# Autodesk Inventor assembly: wahacz_tylny_final
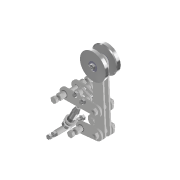
[picture p0: Inventor's stored thumbnail of the model, 180x180]
Saved by Autodesk Inventor 2020.3 (Build 243373000, 373)
## iProperties
Created: 2021-10-24
Part Number: wahacz_tylny_final
Document SubType Name: Assembly
Designer: patry
Author: patry
## Documents named in this file (25)
- C:\Users\patry\Desktop\Semestr 7\Inzynierka\Projekt inventor\Ariadna_inzynierka\Workspaces\Obszar roboczy\Obszar roboczy\Naped\Zawieszenie_v3\wahacz_tylny_final.iam
- C:\Users\patry\Desktop\Semestr 7\Inzynierka\Projekt inventor\Ariadna_inzynierka\Workspaces\Obszar roboczy\Obszar roboczy\Naped\Zawieszenie_v3\ramie_1_wahacza.ipt
- C:\Users\patry\Desktop\Semestr 7\Inzynierka\Projekt inventor\Ariadna_inzynierka\Workspaces\Obszar roboczy\Obszar roboczy\Naped\Zawieszenie_v3\tuleja_TUF106040.ipt
- C:\Users\patry\Desktop\Semestr 7\Inzynierka\Projekt inventor\Ariadna_inzynierka\Workspaces\Obszar roboczy\Obszar roboczy\Naped\Sruby\M6_nut_5mm.ipt
- C:\Users\patry\Desktop\Semestr 7\Inzynierka\Projekt inventor\Ariadna_inzynierka\Workspaces\Obszar roboczy\Obszar roboczy\Naped\Amortyzator\Korpus.ipt
- C:\Users\patry\Desktop\Semestr 7\Inzynierka\Projekt inventor\Ariadna_inzynierka\Workspaces\Obszar roboczy\Obszar roboczy\Naped\Amortyzator\Tlok.ipt
- C:\Users\patry\Desktop\Semestr 7\Inzynierka\Projekt inventor\Ariadna_inzynierka\Workspaces\Obszar roboczy\Obszar roboczy\Naped\Amortyzator\Nakretka.ipt
- C:\Users\patry\Desktop\Semestr 7\Inzynierka\Projekt inventor\Ariadna_inzynierka\Workspaces\Obszar roboczy\Obszar roboczy\Naped\Sruby\M5_nut_5mm.ipt
- C:\Users\patry\Desktop\Semestr 7\Inzynierka\Projekt inventor\Ariadna_inzynierka\Workspaces\Obszar roboczy\Obszar roboczy\Naped\Sruby\M5_70_shaft.ipt
- C:\Users\patry\Desktop\Semestr 7\Inzynierka\Projekt inventor\Ariadna_inzynierka\Workspaces\Obszar roboczy\Obszar roboczy\Naped\Sruby\M3_16_shaft.ipt
- C:\Users\patry\Desktop\Semestr 7\Inzynierka\Projekt inventor\Ariadna_inzynierka\Workspaces\Obszar roboczy\Obszar roboczy\Naped\Sruby\M3_nut_2,5mm.ipt
- C:\Users\patry\Desktop\Semestr 7\Inzynierka\Projekt inventor\Ariadna_inzynierka\Workspaces\Obszar roboczy\Obszar roboczy\Naped\Zawieszenie_v3\wspornik_amortyzatora.ipt
- C:\Users\patry\Desktop\Semestr 7\Inzynierka\Projekt inventor\Ariadna_inzynierka\Workspaces\Obszar roboczy\Obszar roboczy\Naped\Sruby\M6_40_shaft.ipt
- C:\Users\patry\Desktop\Semestr 7\Inzynierka\Projekt inventor\Ariadna_inzynierka\Workspaces\Obszar roboczy\Obszar roboczy\Naped\Sruby\tuleja_M6_M10_7.ipt
- C:\Users\patry\Desktop\Semestr 7\Inzynierka\Projekt inventor\Ariadna_inzynierka\Workspaces\Obszar roboczy\Obszar roboczy\Naped\Sruby\M6_1,25_pad.ipt
- C:\Users\patry\Desktop\Semestr 7\Inzynierka\Projekt inventor\Ariadna_inzynierka\Workspaces\Obszar roboczy\Obszar roboczy\Naped\Sruby\M6_70_shaft.ipt
- C:\Users\patry\Desktop\Semestr 7\Inzynierka\Projekt inventor\Ariadna_inzynierka\Workspaces\Obszar roboczy\Obszar roboczy\Naped\Sruby\M5_40_shaft.ipt
- M5_shaft.ipt
- C:\Users\patry\Desktop\Semestr 7\Inzynierka\Projekt inventor\Ariadna_inzynierka\Workspaces\Obszar roboczy\Obszar roboczy\Naped\Sruby\tuleja_M5_M9_4,5.ipt
- C:\Users\patry\Desktop\Semestr 7\Inzynierka\Projekt inventor\Ariadna_inzynierka\Workspaces\Obszar roboczy\Obszar roboczy\Naped\Zawieszenie_v3\glowny_wahacz_zewn.ipt
- C:\Users\patry\Desktop\Semestr 7\Inzynierka\Projekt inventor\Ariadna_inzynierka\Workspaces\Obszar roboczy\Obszar roboczy\Naped\Zawieszenie_v3\independent_wheel_pair.iam
- C:\Users\patry\Desktop\Semestr 7\Inzynierka\Projekt inventor\Ariadna_inzynierka\Workspaces\Obszar roboczy\Obszar roboczy\Naped\Sruby\tuleja_M6_M10_6.ipt
- C:\Users\patry\Desktop\Semestr 7\Inzynierka\Projekt inventor\Ariadna_inzynierka\Workspaces\Obszar roboczy\Obszar roboczy\Naped\Sruby\tuleja_M5_M9_17.5.ipt
- C:\Users\patry\Desktop\Semestr 7\Inzynierka\Projekt inventor\Ariadna_inzynierka\Workspaces\Obszar roboczy\Obszar roboczy\Naped\Zawieszenie_v3\ramie_2_wahacza_tylnego.ipt
- C:\Users\patry\Desktop\Semestr 7\Inzynierka\Projekt inventor\Ariadna_inzynierka\Workspaces\Obszar roboczy\Obszar roboczy\Naped\Sruby\M6x25_plaski_leb.ipt
## Components (72 placed, 23 different names)
1. ramie_1_wahacza:1 — Zestawiające:7, Zestawiające:8, Kątowe:4, Zestawiające:108, Zestawiające:109, Zestawiające:110, Równoległe:6, Zestawiające:114, Zestawiające:158, Równoległe:11, Zestawiające:159, Równoległe:12, Zestawiające:161, Zestawiające:163, Zestawiające:175, Zestawiające:179, Zestawiające:203, Zestawiające:204
2. tuleja_TUF106040:1 — Zestawiające:93, Zestawiające:200, Zestawiające:250, Zestawiające:251
3. tuleja_TUF106040:2 — Zestawiające:238, Zestawiające:252, Zestawiające:253, Zestawiające:257, Zestawiające:267
4. tuleja_TUF106040:3 — Zestawiające:202, Zestawiające:203, Zestawiające:204
5. tuleja_TUF106040:4 — Zestawiające:7, Zestawiające:8, Kątowe:4, Zestawiające:111, Zestawiające:132
6. tuleja_TUF106040:5 — Zestawiające:89, Zestawiające:201, Zestawiające:240
7. tuleja_TUF106040:6 — Zestawiające:88, Zestawiające:90, Zestawiające:189, Zestawiające:198
8. tuleja_TUF106040:7 — Zestawiające:93, Zestawiające:112, Zestawiające:140, Zestawiające:258, Zestawiające:259
9. tuleja_TUF106040:8 — Zestawiające:236, Zestawiające:260, Zestawiające:261, Zestawiające:262
10. M6_nut_5mm:2 — Zestawiające:113, Zestawiające:114
11. Korpus:1 — Walcowe:1, Zestawiające:83, Równoległe:4, Zestawiające:87, Zestawiające:248
12. Tlok:1 — Walcowe:1, Zestawiające:102, Zestawiające:103
13. Nakretka:1
14. M5_nut_5mm:1 — Zestawiające:84, Zestawiające:86, Zestawiające:87, Równoległe:9, Równoległe:10, Zestawiające:242
15. M5_70_shaft:1 — Zestawiające:83, Równoległe:4, Zestawiające:84, Zestawiające:85, Równoległe:8, Zestawiające:241, Zestawiające:243, Zestawiające:245, Zestawiające:247
16. ramie_1_wahacza:3 — Zestawiające:88, Zestawiające:89, Zestawiające:90, Zestawiające:116, Zestawiające:165, Zestawiające:167, Zestawiające:173, Zestawiające:177, Zestawiające:201, Zestawiające:224
17. M5_nut_5mm:2 — Zestawiające:85, Zestawiające:86, Zestawiające:244
18. M3_16_shaft:1 — Zestawiające:97, Równoległe:5, Zestawiające:98, Zestawiające:100, Zestawiające:102
19. M3_nut_2,5mm:1 — Zestawiające:98, Zestawiające:99
20. M3_nut_2,5mm:2 — Zestawiające:100, Zestawiające:101
21. wspornik_amortyzatora:1 — Zestawiające:94, Zestawiające:95, Zestawiające:96, Równoległe:5, Zestawiające:99, Zestawiające:108, Zestawiające:109, Zestawiające:110
22. wspornik_amortyzatora:2 — Zestawiające:94, Zestawiające:95, Zestawiające:96, Zestawiające:97, Zestawiające:101, Zestawiające:103
23. M6_40_shaft:1 — Zestawiające:111, Równoległe:6, Zestawiające:113, Zestawiające:115, Zestawiające:121, Zestawiające:127, Zestawiające:131, Zestawiające:182, Zestawiające:186, Zestawiające:189
24. M6_40_shaft:2 — Zestawiające:112, Zestawiające:117, Zestawiające:119, Zestawiające:123, Zestawiające:135, Zestawiające:139, Zestawiające:180, Zestawiające:185, Równoległe:13
25. M6_nut_5mm:11 — Zestawiające:115, Zestawiające:116
26. M6_nut_5mm:12 — Zestawiające:117, Zestawiające:270, Równoległe:13
27. M6_nut_5mm:13 — Zestawiające:119, Zestawiające:269
28. tuleja_M6_M10_7:1 — Zestawiające:121, Zestawiające:196
29. tuleja_M6_M10_7:2 — Zestawiające:123, Zestawiające:181
30. M6_1,25_pad:1 — Zestawiające:125, Zestawiające:126, Zestawiające:127, Zestawiające:197
31. M6_1,25_pad:2 — Zestawiające:125, Zestawiające:126, Zestawiające:198
32. M6_1,25_pad:3 — Zestawiające:131, Zestawiające:132
33. M6_1,25_pad:4 — Zestawiające:194
34. M6_1,25_pad:5 — Zestawiające:135, Zestawiające:199
35. M6_1,25_pad:6 — Zestawiające:200
36. M6_1,25_pad:7 — Zestawiające:139, Zestawiające:140
37. M6_1,25_pad:8 — Zestawiające:195
38. M6_70_shaft:2 — Równoległe:8, Zestawiające:144, Zestawiające:145, Zestawiające:202, Zestawiające:229, Zestawiające:231, Zestawiające:233, Zestawiające:239
39. M6_nut_5mm:14 — Zestawiające:144, Zestawiające:146, Zestawiające:230
40. M6_nut_5mm:15 — Zestawiające:145, Zestawiające:146, Równoległe:9, Zestawiające:232
41. M6_nut_5mm:16 — Zestawiające:148, Zestawiające:228, Zestawiające:264
42. M6_nut_5mm:17 — Zestawiające:148, Równoległe:10, Zestawiające:226, Zestawiające:254, Zestawiające:255
43. M5_shaft:1 — Zestawiające:158, Równoległe:11, Zestawiające:162, Zestawiające:164, Zestawiające:172, Zestawiające:174
44. M5_shaft:2 — Zestawiające:159, Równoległe:12, Zestawiające:160, Zestawiające:166, Zestawiające:176, Zestawiające:178, Zestawiające:224
45. M5_nut_5mm:3 — Zestawiające:160, Zestawiające:161
46. M5_nut_5mm:4 — Zestawiające:162, Zestawiające:163
47. M5_nut_5mm:5 — Zestawiające:164, Zestawiające:165
48. M5_nut_5mm:6 — Zestawiające:166, Zestawiające:167
49. tuleja_M5_M9_4,5:1 — Zestawiające:172, Zestawiające:173
50. tuleja_M5_M9_4,5:2 — Zestawiające:174, Zestawiające:175
51. tuleja_M5_M9_4,5:3 — Zestawiające:176, Zestawiające:177
52. tuleja_M5_M9_4,5:4 — Zestawiające:178, Zestawiające:179
53. glowny_wahacz_zewn:1 — Zestawiające:180, Zestawiające:181, Zestawiające:182, Zestawiające:196, Zestawiające:197, Zestawiające:199, Zestawiające:249
54. glowny_wahacz_zewn:2 — Zestawiające:185, Zestawiające:186, Zestawiające:194, Zestawiające:195, Zestawiające:221, Zestawiające:222, Zestawiające:223
55. independent_wheel_pair:1 [sub-assembly] — Zestawiające:221, Zestawiające:222, Zestawiające:249
56. tuleja_M6_M10_7:3 — Zestawiające:223
57. tuleja_M6_M10_6:1 — Zestawiające:233, Zestawiające:234
58. M6_nut_5mm:18 — Zestawiające:226, Zestawiające:254, Zestawiające:255, Zestawiające:256, Zestawiające:257
59. M6_nut_5mm:19 — Zestawiające:228, Zestawiające:263, Zestawiające:264, Zestawiające:265
60. M6_nut_5mm:20 — Zestawiające:229, Zestawiające:230, Zestawiające:234
61. M6_nut_5mm:21 — Zestawiające:231, Zestawiające:232
62. tuleja_M6_M10_6:2 — Zestawiające:236, Zestawiające:262, Zestawiające:263
63. tuleja_M6_M10_6:3 — Zestawiające:238, Zestawiające:256
64. tuleja_M6_M10_6:4 — Zestawiające:239, Zestawiające:240
65. M5_nut_5mm:7 — Zestawiające:241, Zestawiające:242
66. M5_nut_5mm:8 — Zestawiające:243, Zestawiające:244, Zestawiające:246
67. tuleja_M5_M9_17.5:1 — Zestawiające:247, Zestawiające:248
68. tuleja_M5_M9_17.5:2 — Zestawiające:245, Zestawiające:246
69. ramie_2_wahacza_tylnego:1 — Zestawiające:250, Zestawiające:251, Zestawiające:252, Zestawiające:253, Zestawiające:268, Zestawiające:270
70. ramie_2_wahacza_tylnego:2 — Zestawiające:258, Zestawiające:259, Zestawiające:260, Zestawiające:261, Zestawiające:266, Zestawiające:269
71. M6x25_plaski_leb:1 — Zestawiające:267, Zestawiające:268
72. M6x25_plaski_leb:2 — Zestawiające:265, Zestawiające:266
## Relationships (150: Mate 138, Flush 9, Angle 2, CylindricalJoint 1)
- Zestawiające:7 [Mate]: ramie_1_wahacza:1 ↔ tuleja_TUF106040:4
- Zestawiające:8 [Mate]: ramie_1_wahacza:1 ↔ tuleja_TUF106040:4
- Kątowe:4 [Angle] (0 deg): ramie_1_wahacza:1 ↔ tuleja_TUF106040:4
- [Mate]: Korpus:1 ↔ Tlok:1
- [Angle] (0 deg): Korpus:1 ↔ Tlok:1
- [Mate]: Korpus:1 ↔ Nakretka:1
- [Mate] (5 mm): Korpus:1 ↔ Nakretka:1
- Walcowe:1 [CylindricalJoint]: Korpus:1 ↔ Tlok:1
- Zestawiające:83 [Mate]: Korpus:1 ↔ M5_70_shaft:1
- Równoległe:4 [Flush] (-32.5 mm): Korpus:1 ↔ M5_70_shaft:1
- Zestawiające:84 [Mate]: M5_nut_5mm:1 ↔ M5_70_shaft:1
- Zestawiające:85 [Mate]: M5_70_shaft:1 ↔ M5_nut_5mm:2
- Zestawiające:86 [Mate] (60 mm): M5_nut_5mm:1 ↔ M5_nut_5mm:2
- Zestawiające:87 [Mate] (27.5 mm): Korpus:1 ↔ M5_nut_5mm:1
- Zestawiające:88 [Mate]: tuleja_TUF106040:6 ↔ ramie_1_wahacza:3
- Zestawiające:89 [Mate]: tuleja_TUF106040:5 ↔ ramie_1_wahacza:3
- Zestawiające:90 [Mate]: tuleja_TUF106040:6 ↔ ramie_1_wahacza:3
- Zestawiające:93 [Mate]: tuleja_TUF106040:1 ↔ tuleja_TUF106040:7
- Zestawiające:94 [Mate]: wspornik_amortyzatora:1 ↔ wspornik_amortyzatora:2
- Zestawiające:95 [Mate]: wspornik_amortyzatora:1 ↔ wspornik_amortyzatora:2
- Zestawiające:96 [Mate] (5 mm): wspornik_amortyzatora:1 ↔ wspornik_amortyzatora:2
- Zestawiające:97 [Mate]: M3_16_shaft:1 ↔ wspornik_amortyzatora:2
- Równoległe:5 [Flush] (-2.5 mm): M3_16_shaft:1 ↔ wspornik_amortyzatora:1
- Zestawiające:98 [Mate]: M3_16_shaft:1 ↔ M3_nut_2,5mm:1
- Zestawiające:99 [Mate]: M3_nut_2,5mm:1 ↔ wspornik_amortyzatora:1
- Zestawiające:100 [Mate]: M3_16_shaft:1 ↔ M3_nut_2,5mm:2
- Zestawiające:101 [Mate]: M3_nut_2,5mm:2 ↔ wspornik_amortyzatora:2
- Zestawiające:102 [Mate]: Tlok:1 ↔ M3_16_shaft:1
- Zestawiające:103 [Mate]: Tlok:1 ↔ wspornik_amortyzatora:2
- Zestawiające:108 [Mate]: ramie_1_wahacza:1 ↔ wspornik_amortyzatora:1
- Zestawiające:109 [Mate]: ramie_1_wahacza:1 ↔ wspornik_amortyzatora:1
- Zestawiające:110 [Mate] (4.5 mm): ramie_1_wahacza:1 ↔ wspornik_amortyzatora:1
- Zestawiające:111 [Mate]: tuleja_TUF106040:4 ↔ M6_40_shaft:1
- Równoległe:6 [Flush] (7 mm): ramie_1_wahacza:1 ↔ M6_40_shaft:1
- Zestawiające:112 [Mate]: tuleja_TUF106040:7 ↔ M6_40_shaft:2
- Zestawiające:113 [Mate]: M6_nut_5mm:2 ↔ M6_40_shaft:1
- Zestawiające:114 [Mate]: ramie_1_wahacza:1 ↔ M6_nut_5mm:2
- Zestawiające:115 [Mate]: M6_40_shaft:1 ↔ M6_nut_5mm:11
- Zestawiające:116 [Mate]: ramie_1_wahacza:3 ↔ M6_nut_5mm:11
- Zestawiające:117 [Mate]: M6_40_shaft:2 ↔ M6_nut_5mm:12
- Zestawiające:119 [Mate]: M6_40_shaft:2 ↔ M6_nut_5mm:13
- Zestawiające:121 [Mate]: M6_40_shaft:1 ↔ tuleja_M6_M10_7:1
- Zestawiające:123 [Mate]: M6_40_shaft:2 ↔ tuleja_M6_M10_7:2
- Zestawiające:125 [Mate]: M6_1,25_pad:1 ↔ M6_1,25_pad:2
- Zestawiające:126 [Mate]: M6_1,25_pad:1 ↔ M6_1,25_pad:2
- Zestawiające:127 [Mate]: M6_40_shaft:1 ↔ M6_1,25_pad:1
- [Mate]: M6_1,25_pad:3 ↔ M6_1,25_pad:4
- [Mate]: M6_1,25_pad:3 ↔ M6_1,25_pad:4
- Zestawiające:131 [Mate]: M6_40_shaft:1 ↔ M6_1,25_pad:3
- Zestawiające:132 [Mate]: tuleja_TUF106040:4 ↔ M6_1,25_pad:3
- [Mate]: M6_1,25_pad:5 ↔ M6_1,25_pad:6
- [Mate]: M6_1,25_pad:5 ↔ M6_1,25_pad:6
- Zestawiające:135 [Mate]: M6_40_shaft:2 ↔ M6_1,25_pad:5
- [Mate]: M6_1,25_pad:7 ↔ M6_1,25_pad:8
- [Mate]: M6_1,25_pad:7 ↔ M6_1,25_pad:8
- Zestawiające:139 [Mate]: M6_40_shaft:2 ↔ M6_1,25_pad:7
- Zestawiające:140 [Mate]: tuleja_TUF106040:7 ↔ M6_1,25_pad:7
- Równoległe:8 [Flush]: M5_70_shaft:1 ↔ M6_70_shaft:2
- Zestawiające:144 [Mate]: M6_70_shaft:2 ↔ M6_nut_5mm:14
- Zestawiające:145 [Mate]: M6_70_shaft:2 ↔ M6_nut_5mm:15
- Zestawiające:146 [Mate] (60 mm): M6_nut_5mm:14 ↔ M6_nut_5mm:15
- Równoległe:9 [Flush]: M5_nut_5mm:1 ↔ M6_nut_5mm:15
- [Mate] (60 mm): M6_nut_5mm:16 ↔ M6_nut_5mm:17
- Zestawiające:148 [Mate]: M6_nut_5mm:16 ↔ M6_nut_5mm:17
- Równoległe:10 [Flush]: M5_nut_5mm:1 ↔ M6_nut_5mm:17
- Zestawiające:158 [Mate]: ramie_1_wahacza:1 ↔ M5_shaft:1
- Równoległe:11 [Flush] (7 mm): ramie_1_wahacza:1 ↔ M5_shaft:1
- Zestawiające:159 [Mate]: ramie_1_wahacza:1 ↔ M5_shaft:2
- Równoległe:12 [Flush] (7 mm): ramie_1_wahacza:1 ↔ M5_shaft:2
- Zestawiające:160 [Mate]: M5_shaft:2 ↔ M5_nut_5mm:3
- Zestawiające:161 [Mate]: ramie_1_wahacza:1 ↔ M5_nut_5mm:3
- Zestawiające:162 [Mate]: M5_shaft:1 ↔ M5_nut_5mm:4
- Zestawiające:163 [Mate]: ramie_1_wahacza:1 ↔ M5_nut_5mm:4
- Zestawiające:164 [Mate]: M5_shaft:1 ↔ M5_nut_5mm:5
- Zestawiające:165 [Mate]: ramie_1_wahacza:3 ↔ M5_nut_5mm:5
- Zestawiające:166 [Mate]: M5_shaft:2 ↔ M5_nut_5mm:6
- Zestawiające:167 [Mate]: ramie_1_wahacza:3 ↔ M5_nut_5mm:6
- Zestawiające:172 [Mate]: M5_shaft:1 ↔ tuleja_M5_M9_4,5:1
- Zestawiające:173 [Mate]: ramie_1_wahacza:3 ↔ tuleja_M5_M9_4,5:1
- Zestawiające:174 [Mate]: M5_shaft:1 ↔ tuleja_M5_M9_4,5:2
- Zestawiające:175 [Mate]: ramie_1_wahacza:1 ↔ tuleja_M5_M9_4,5:2
- Zestawiające:176 [Mate]: M5_shaft:2 ↔ tuleja_M5_M9_4,5:3
- Zestawiające:177 [Mate]: ramie_1_wahacza:3 ↔ tuleja_M5_M9_4,5:3
- Zestawiające:178 [Mate]: M5_shaft:2 ↔ tuleja_M5_M9_4,5:4
- Zestawiające:179 [Mate]: ramie_1_wahacza:1 ↔ tuleja_M5_M9_4,5:4
- Zestawiające:180 [Mate]: M6_40_shaft:2 ↔ glowny_wahacz_zewn:1
- Zestawiające:181 [Mate]: tuleja_M6_M10_7:2 ↔ glowny_wahacz_zewn:1
- Zestawiające:182 [Mate]: M6_40_shaft:1 ↔ glowny_wahacz_zewn:1
- Zestawiające:185 [Mate]: M6_40_shaft:2 ↔ glowny_wahacz_zewn:2
- Zestawiające:186 [Mate]: M6_40_shaft:1 ↔ glowny_wahacz_zewn:2
- Zestawiające:189 [Mate]: tuleja_TUF106040:6 ↔ M6_40_shaft:1
- Zestawiające:194 [Mate]: M6_1,25_pad:4 ↔ glowny_wahacz_zewn:2
- Zestawiające:195 [Mate]: M6_1,25_pad:8 ↔ glowny_wahacz_zewn:2
- Zestawiające:196 [Mate]: tuleja_M6_M10_7:1 ↔ glowny_wahacz_zewn:1
- Zestawiające:197 [Mate]: M6_1,25_pad:1 ↔ glowny_wahacz_zewn:1
- Zestawiające:198 [Mate]: tuleja_TUF106040:6 ↔ M6_1,25_pad:2
- Zestawiające:199 [Mate]: M6_1,25_pad:5 ↔ glowny_wahacz_zewn:1
- Zestawiające:200 [Mate]: tuleja_TUF106040:1 ↔ M6_1,25_pad:6
- Zestawiające:201 [Mate]: tuleja_TUF106040:5 ↔ ramie_1_wahacza:3
- Zestawiające:202 [Mate]: tuleja_TUF106040:3 ↔ M6_70_shaft:2
- Zestawiające:203 [Mate]: ramie_1_wahacza:1 ↔ tuleja_TUF106040:3
- Zestawiające:204 [Mate]: ramie_1_wahacza:1 ↔ tuleja_TUF106040:3
- [Mate]: independent_wheel_pair:1 ↔ tuleja_M6_M10_7:3
- Zestawiające:221 [Mate]: glowny_wahacz_zewn:2 ↔ independent_wheel_pair:1
- Zestawiające:222 [Mate]: glowny_wahacz_zewn:2 ↔ independent_wheel_pair:1
- Zestawiające:223 [Mate]: glowny_wahacz_zewn:2 ↔ tuleja_M6_M10_7:3
- Zestawiające:224 [Mate]: ramie_1_wahacza:3 ↔ M5_shaft:2
- Zestawiające:226 [Mate] (5 mm): M6_nut_5mm:17 ↔ M6_nut_5mm:18
- Zestawiające:228 [Mate] (5 mm): M6_nut_5mm:16 ↔ M6_nut_5mm:19
- Zestawiające:229 [Mate]: M6_70_shaft:2 ↔ M6_nut_5mm:20
- Zestawiające:230 [Mate] (5 mm): M6_nut_5mm:14 ↔ M6_nut_5mm:20
- Zestawiające:231 [Mate]: M6_70_shaft:2 ↔ M6_nut_5mm:21
- Zestawiające:232 [Mate] (5 mm): M6_nut_5mm:15 ↔ M6_nut_5mm:21
- Zestawiające:233 [Mate]: M6_70_shaft:2 ↔ tuleja_M6_M10_6:1
- Zestawiające:234 [Mate]: tuleja_M6_M10_6:1 ↔ M6_nut_5mm:20
- Zestawiające:236 [Mate]: tuleja_TUF106040:8 ↔ tuleja_M6_M10_6:2
- Zestawiające:238 [Mate]: tuleja_TUF106040:2 ↔ tuleja_M6_M10_6:3
- Zestawiające:239 [Mate]: M6_70_shaft:2 ↔ tuleja_M6_M10_6:4
- Zestawiające:240 [Mate]: tuleja_TUF106040:5 ↔ tuleja_M6_M10_6:4
- Zestawiające:241 [Mate]: M5_70_shaft:1 ↔ M5_nut_5mm:7
- Zestawiające:242 [Mate] (5 mm): M5_nut_5mm:1 ↔ M5_nut_5mm:7
- Zestawiające:243 [Mate]: M5_70_shaft:1 ↔ M5_nut_5mm:8
- Zestawiające:244 [Mate] (5 mm): M5_nut_5mm:2 ↔ M5_nut_5mm:8
- Zestawiające:245 [Mate]: M5_70_shaft:1 ↔ tuleja_M5_M9_17.5:2
- Zestawiające:246 [Mate]: M5_nut_5mm:8 ↔ tuleja_M5_M9_17.5:2
- Zestawiające:247 [Mate]: M5_70_shaft:1 ↔ tuleja_M5_M9_17.5:1
- Zestawiające:248 [Mate]: Korpus:1 ↔ tuleja_M5_M9_17.5:1
- Zestawiające:249 [Mate]: glowny_wahacz_zewn:1 ↔ independent_wheel_pair:1
- Zestawiające:250 [Mate]: tuleja_TUF106040:1 ↔ ramie_2_wahacza_tylnego:1
- Zestawiające:251 [Mate]: tuleja_TUF106040:1 ↔ ramie_2_wahacza_tylnego:1
- Zestawiające:252 [Mate]: tuleja_TUF106040:2 ↔ ramie_2_wahacza_tylnego:1
- Zestawiające:253 [Mate]: tuleja_TUF106040:2 ↔ ramie_2_wahacza_tylnego:1
- Zestawiające:254 [Mate]: M6_nut_5mm:17 ↔ M6_nut_5mm:18
- Zestawiające:255 [Mate] (5 mm): M6_nut_5mm:17 ↔ M6_nut_5mm:18
- Zestawiające:256 [Mate]: M6_nut_5mm:18 ↔ tuleja_M6_M10_6:3
- Zestawiające:257 [Mate]: tuleja_TUF106040:2 ↔ M6_nut_5mm:18
- Zestawiające:258 [Mate]: tuleja_TUF106040:7 ↔ ramie_2_wahacza_tylnego:2
- Zestawiające:259 [Mate]: tuleja_TUF106040:7 ↔ ramie_2_wahacza_tylnego:2
- Zestawiające:260 [Mate]: tuleja_TUF106040:8 ↔ ramie_2_wahacza_tylnego:2
- Zestawiające:261 [Mate]: tuleja_TUF106040:8 ↔ ramie_2_wahacza_tylnego:2
- Zestawiające:262 [Mate]: tuleja_TUF106040:8 ↔ tuleja_M6_M10_6:2
- Zestawiające:263 [Mate]: M6_nut_5mm:19 ↔ tuleja_M6_M10_6:2
- Zestawiające:264 [Mate]: M6_nut_5mm:16 ↔ M6_nut_5mm:19
- Zestawiające:265 [Mate]: M6_nut_5mm:19 ↔ M6x25_plaski_leb:2
- Zestawiające:266 [Mate]: ramie_2_wahacza_tylnego:2 ↔ M6x25_plaski_leb:2
- Zestawiające:267 [Mate]: tuleja_TUF106040:2 ↔ M6x25_plaski_leb:1
- Zestawiające:268 [Mate]: ramie_2_wahacza_tylnego:1 ↔ M6x25_plaski_leb:1
- Zestawiające:269 [Mate]: M6_nut_5mm:13 ↔ ramie_2_wahacza_tylnego:2
- Zestawiające:270 [Mate]: M6_nut_5mm:12 ↔ ramie_2_wahacza_tylnego:1
- Równoległe:13 [Flush] (-2 mm): M6_40_shaft:2 ↔ M6_nut_5mm:12
## Named parameters: d83_d6 = 0 mm, d84_d7 = 0 mm, d85_d8 = -13 mm, d86_d0 = 0 mm, d87_d1 = 0 deg, d88_d3 = 0 mm, d89_d4 = 5 mm, d90_d5 = 0 deg, d158_d154 = 0 mm, d159_d155 = 0 mm, d162_d154 = 0 mm, d163_d155 = 0 mm, d166_d154 = 0 mm, d167_d155 = 0 mm, d178_d176 = 60 mm
